# Autodesk Inventor assembly: NP18-12
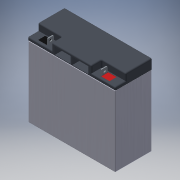
[picture p0: Inventor's stored thumbnail of the model, 180x180]
Saved by Autodesk Inventor 2016 (Build 200138000, 138)
## iProperties
Category: Electrical
Company: Autodesk Inc.
Created: 2013-12-19
Part Number: NP18-12
Document SubType Name: Assembly
Designer: Autodesk
Description: Battery, ,12 volt, 18 AH, Non-spillable
Mass: 6259.57 g
Author: Autodesk Inc.
## Documents named in this file (4)
- C:\Users\FIRSTUser\Documents\GrabCAD\2016 Robot\Imported Components\Electronics\ELEC_Battery_NP18-12B.iam
- C:\Users\Evan\Documents\Robotics\CAD\KOP\Electrical\Parts\Electrical_Yuasa_NP18-12_Top.ipt
- C:\Users\Evan\Documents\Robotics\CAD\KOP\Electrical\Parts\Electrical_Yuasa_Np18-12_Middle.ipt
- C:\Users\FIRSTUser\Documents\GrabCAD\2016 Robot\Imported Components\Electronics\ELEC_Battery_NP18-12B_SUB.ipt
## Components (3 placed, 3 different names)
1. Electrical_Yuasa_NP18-12_Top:1 — Flush:1
2. Electrical_Yuasa_Np18-12_Middle:1 — Flush:1
3. ELEC_Battery_NP18-12B_SUB:1
## Relationships (1: Flush 1)
- Flush:1: Electrical_Yuasa_NP18-12_Top:1 ↔ Electrical_Yuasa_Np18-12_Middle:1
